# Autodesk Inventor assembly: 0002_Part_Khop_tay_B
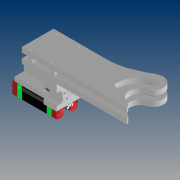
[picture p0: Inventor's stored thumbnail of the model, 180x180]
Saved by Autodesk Inventor 2021 (Build 250183000, 183)
## iProperties
Created: 2024-04-08
Part Number: 0002_Part_Khop_tay_B
Document SubType Name: Assembly
Designer: Admin
Author: Admin
## Documents named in this file (4)
- C:\Users\Admin\Desktop\DO_AN_TOT_NGHIEP_2024\Mechanical\Design_in_3D\Version_2\0002_Part_Khop_tay_B.iam
- C:\Users\Admin\Desktop\DO_AN_TOT_NGHIEP_2024\Mechanical\Design_in_3D\Version_1\0012_Bo_truot.iam
- C:\Users\Admin\Desktop\DO_AN_TOT_NGHIEP_2024\Mechanical\Design_in_3D\Version_1\16_Khau_hai.ipt
- C:\Users\Admin\Desktop\DO_AN_TOT_NGHIEP_2024\Mechanical\Design_in_3D\Version_1\21_Tam_go_trung_gian.ipt
## Components (3 placed, 3 different names)
1. 0012_Bo_truot:1 [sub-assembly] — Insert:1, Mate:1
2. 16_Khau_hai:1 — Insert:2
3. 21_Tam_go_trung_gian:1 — Insert:1, Mate:1, Insert:2
## Relationships (4: Insert 2, Flush 1, Mate 1)
- [Flush]: 0012_Bo_truot:1 ↔ 16_Khau_hai:1
- Insert:1: 0012_Bo_truot:1 ↔ 21_Tam_go_trung_gian:1
- Mate:1: 0012_Bo_truot:1 ↔ 21_Tam_go_trung_gian:1
- Insert:2: 16_Khau_hai:1 ↔ 21_Tam_go_trung_gian:1
